# Autodesk Inventor assembly: Intake motor on xrail
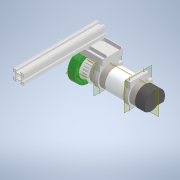
[picture p0: Inventor's stored thumbnail of the model, 180x180]
Saved by Autodesk Inventor 2020 (Build 240168000, 168)
## iProperties
Created: 2020-01-13
Part Number: Intake motor on xrail
Document SubType Name: Assembly
Designer: ball
Author: ball
## Documents named in this file (5)
- D:\FTC8863\2019 Robot\Collection\Intake motor on xrail.iam
- D:\FTC8863\2019 Robot\Collection\neverest 40 + mounts.iam
- D:\FTC8863\2019 Robot\Collection\intake motor mount to xrail.ipt
- D:\FTC8863\Actobotics\565 parts\565030.ipt
- D:\FTC8863\2019 Robot\general robot componets\pulley .25 in + wheel.2.iam
## Components (4 placed, 4 different names)
1. neverest 40 + mounts:1 [sub-assembly] — Flush:3, Mate:5, Mate:6
2. 565030:1 — Flush:4
3. intake motor mount to xrail:1 — Flush:3, Flush:4
4. pulley .25 in + wheel.2:1 [sub-assembly] — Mate:5, Mate:6
## Relationships (7: Mate 4, Flush 3)
- [Mate]: 565030:1 ↔ intake motor mount to xrail:1
- [Flush]: 565030:1 ↔ intake motor mount to xrail:1
- [Mate]: neverest 40 + mounts:1 ↔ intake motor mount to xrail:1
- Flush:3 (-5.08 mm): neverest 40 + mounts:1 ↔ intake motor mount to xrail:1
- Flush:4: 565030:1 ↔ intake motor mount to xrail:1
- Mate:5: neverest 40 + mounts:1 ↔ pulley .25 in + wheel.2:1
- Mate:6: neverest 40 + mounts:1 ↔ pulley .25 in + wheel.2:1
